# Autodesk Inventor assembly: assembly
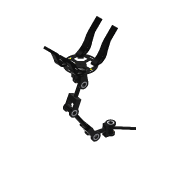
[picture p0: Inventor's stored thumbnail of the model, 180x180]
Saved by Autodesk Inventor 2018 (Build 220112000, 112)
## iProperties
Created: 2017-11-18
Part Number: assembly
Document SubType Name: Assembly
Designer: Bardo91
Author: Bardo91
## Documents named in this file (11)
- E:\programming\cad_hexacopter\positioner\NewVersion\assembly.iam
- E:\programming\cad_hexacopter\positioner\NewVersion\Positioner_Fija_BASE_v2.ipt
- E:\programming\cad_hexacopter\positioner\NewVersion\Positioner_Adapter_Der.ipt
- E:\programming\cad_hexacopter\positioner\NewVersion\Positioner_Adapter_Izq.ipt
- E:\programming\cad_hexacopter\positioner\NewVersion\Positioner_BASE_v2.ipt
- E:\programming\cad_hexacopter\positioner\NewVersion\Positioner_2.ipt
- E:\programming\cad_hexacopter\positioner\NewVersion\Positioner_1.ipt
- E:\programming\cad_hexacopter\positioner\NewVersion\Positioner_Rotor_HAND.ipt
- E:\programming\cad_hexacopter\positioner\NewVersion\Positioner_HAND.ipt
- E:\programming\cad_hexacopter\positioner\potentiometer.ipt
- E:\programming\cad_hexacopter\positioner\NewVersion\treat.ipt
## Components (21 placed, 10 different names)
1. Positioner_Fija_BASE_v2:1 — Mate:13, Mate:14, Mate:19, Mate:20, Mate:21, Mate:22, Mate:23, Mate:24, Mate:25, Mate:26, Mate:27, Mate:28, Mate:29, Mate:30
2. Positioner_BASE_v2:1 — Mate:13, Mate:14, Mate:15, Flush:1, Mate:39, Mate:40, Mate:41, Mate:49, Flush:8, Mate:50, Mate:51, Mate:52, Mate:53
3. Positioner_2:1 — Mate:15, Flush:1, Mate:16, Flush:2, Mate:31, Mate:32, Mate:42, Mate:46, Flush:5
4. Positioner_1:1 — Mate:16, Flush:2, Mate:17, Flush:3, Mate:33, Mate:34, Mate:43, Mate:47, Flush:6
5. Positioner_Rotor_HAND:1 — Mate:18, Flush:4, Mate:37, Mate:38, Mate:45
6. Positioner_HAND:1 — Mate:17, Flush:3, Mate:18, Flush:4, Mate:35, Mate:36, Mate:44, Flush:7, Mate:48
7. Positioner_Adapter_Der:1 — Mate:20, Mate:29, Mate:30
8. Positioner_Adapter_Der:2 — Mate:19, Mate:23, Mate:24
9. Positioner_Adapter_Izq:1 — Mate:21, Mate:27, Mate:28
10. Positioner_Adapter_Izq:2 — Mate:22, Mate:25, Mate:26
11. potentiometer:1 — Mate:31, Mate:32, Mate:42
12. potentiometer:2 — Mate:35, Mate:36, Mate:44
13. potentiometer:3 — Mate:33, Mate:34, Mate:43
14. potentiometer:4 — Mate:39, Mate:40, Mate:41
15. potentiometer:5 — Mate:37, Mate:38, Mate:45
16. treat:1 — Mate:46, Flush:5
17. treat:2 — Mate:49, Flush:8
18. treat:3 — Mate:52, Mate:53
19. treat:4 — Mate:50, Mate:51
20. treat:5 — Flush:7, Mate:48
21. treat:6 — Mate:47, Flush:6
## Relationships (49: Mate 41, Flush 8)
- Mate:13 (1 mm): Positioner_Fija_BASE_v2:1 ↔ Positioner_BASE_v2:1
- Mate:14: Positioner_Fija_BASE_v2:1 ↔ Positioner_BASE_v2:1
- Mate:15: Positioner_BASE_v2:1 ↔ Positioner_2:1
- Flush:1: Positioner_BASE_v2:1 ↔ Positioner_2:1
- Mate:16: Positioner_2:1 ↔ Positioner_1:1
- Flush:2: Positioner_2:1 ↔ Positioner_1:1
- Mate:17: Positioner_1:1 ↔ Positioner_HAND:1
- Flush:3: Positioner_1:1 ↔ Positioner_HAND:1
- Mate:18: Positioner_Rotor_HAND:1 ↔ Positioner_HAND:1
- Flush:4: Positioner_Rotor_HAND:1 ↔ Positioner_HAND:1
- Mate:19: Positioner_Fija_BASE_v2:1 ↔ Positioner_Adapter_Der:2
- Mate:20: Positioner_Fija_BASE_v2:1 ↔ Positioner_Adapter_Der:1
- Mate:21: Positioner_Fija_BASE_v2:1 ↔ Positioner_Adapter_Izq:1
- Mate:22: Positioner_Fija_BASE_v2:1 ↔ Positioner_Adapter_Izq:2
- Mate:23: Positioner_Fija_BASE_v2:1 ↔ Positioner_Adapter_Der:2
- Mate:24: Positioner_Fija_BASE_v2:1 ↔ Positioner_Adapter_Der:2
- Mate:25: Positioner_Fija_BASE_v2:1 ↔ Positioner_Adapter_Izq:2
- Mate:26: Positioner_Fija_BASE_v2:1 ↔ Positioner_Adapter_Izq:2
- Mate:27: Positioner_Fija_BASE_v2:1 ↔ Positioner_Adapter_Izq:1
- Mate:28: Positioner_Fija_BASE_v2:1 ↔ Positioner_Adapter_Izq:1
- Mate:29: Positioner_Fija_BASE_v2:1 ↔ Positioner_Adapter_Der:1
- Mate:30: Positioner_Fija_BASE_v2:1 ↔ Positioner_Adapter_Der:1
- Mate:31 (0.5 mm): Positioner_2:1 ↔ potentiometer:1
- Mate:32: Positioner_2:1 ↔ potentiometer:1
- Mate:33 (0.5 mm): Positioner_1:1 ↔ potentiometer:3
- Mate:34: Positioner_1:1 ↔ potentiometer:3
- Mate:35 (0.5 mm): Positioner_HAND:1 ↔ potentiometer:2
- Mate:36: Positioner_HAND:1 ↔ potentiometer:2
- Mate:37 (0.5 mm): Positioner_Rotor_HAND:1 ↔ potentiometer:5
- Mate:38: Positioner_Rotor_HAND:1 ↔ potentiometer:5
- Mate:39: Positioner_BASE_v2:1 ↔ potentiometer:4
- Mate:40 (0.5 mm): Positioner_BASE_v2:1 ↔ potentiometer:4
- Mate:41: Positioner_BASE_v2:1 ↔ potentiometer:4
- Mate:42: Positioner_2:1 ↔ potentiometer:1
- Mate:43: Positioner_1:1 ↔ potentiometer:3
- Mate:44: Positioner_HAND:1 ↔ potentiometer:2
- Mate:45: Positioner_Rotor_HAND:1 ↔ potentiometer:5
- Mate:46: Positioner_2:1 ↔ treat:1
- Flush:5: Positioner_2:1 ↔ treat:1
- Mate:47: Positioner_1:1 ↔ treat:6
- Flush:6: Positioner_1:1 ↔ treat:6
- Flush:7: Positioner_HAND:1 ↔ treat:5
- Mate:48: Positioner_HAND:1 ↔ treat:5
- Mate:49: Positioner_BASE_v2:1 ↔ treat:2
- Flush:8: Positioner_BASE_v2:1 ↔ treat:2
- Mate:50: Positioner_BASE_v2:1 ↔ treat:4
- Mate:51: Positioner_BASE_v2:1 ↔ treat:4
- Mate:52: Positioner_BASE_v2:1 ↔ treat:3
- Mate:53: Positioner_BASE_v2:1 ↔ treat:3
